# Autodesk Inventor assembly: 掃地機固定
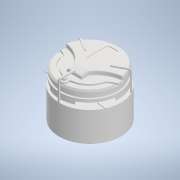
[picture p0: Inventor's stored thumbnail of the model, 180x180]
Saved by Autodesk Inventor 2020 (Build 240168000, 168)
## iProperties
Created: 2021-05-09
Part Number: 掃地機固定
Document SubType Name: Assembly
Designer: User
Author: User
## Documents named in this file (3)
- C:\Users\User\Desktop\stage3-bg1\掃地機固定.iam
- C:\Users\User\Desktop\stage3-bg1\掃地機器人\組合圖2.iam
- C:\Users\User\Desktop\stage3-bg1\掃地機底座.ipt
## Components (2 placed, 2 different names)
1. 組合圖2:1 [sub-assembly] — 角度:1, 相切:1, 相切:2, 貼合:1
2. 掃地機底座:1 — 角度:1, 相切:1, 相切:2, 貼合:1
## Relationships (4: Tangent 2, Angle 1, Mate 1)
- 角度:1 [Angle] (180 deg): 組合圖2:1 ↔ 掃地機底座:1
- 相切:1 [Tangent]: 組合圖2:1 ↔ 掃地機底座:1
- 相切:2 [Tangent]: 組合圖2:1 ↔ 掃地機底座:1
- 貼合:1 [Mate]: 組合圖2:1 ↔ 掃地機底座:1
